# Autodesk Inventor assembly: Lower box main assembly
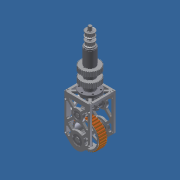
[picture p0: Inventor's stored thumbnail of the model, 180x180]
Saved by Autodesk Inventor 2012 (Build 160160000, 160)
## iProperties
Created: 2012-07-05
Part Number: Lower box main assembly
Document SubType Name: Assembly
Designer: Bryce
Author: Bryce
## Documents named in this file (18)
- C:\Users\Team-2471\Dropbox\Rebound Rumble 2012\Independant Swerves\Inventor 2012\Lower box main assembly.iam
- C:\Users\Team-2471\Dropbox\Rebound Rumble 2012\Independant Swerves\Inventor 2012\lower box side plate.ipt
- C:\Users\Team-2471\Dropbox\Rebound Rumble 2012\Independant Swerves\Inventor 2012\wheel shaft.ipt
- C:\Users\Team-2471\Dropbox\Rebound Rumble 2012\Independant Swerves\Inventor 2012\lower box front plate2.ipt
- C:\Users\Team-2471\Dropbox\Rebound Rumble 2012\Independant Swerves\Imported Components\0.5'' 15 tooth flange.ipt
- C:\Users\Team-2471\Dropbox\Rebound Rumble 2012\Independant Swerves\Inventor 2012\lower box upper shaft.ipt
- C:\Users\Team-2471\Dropbox\Rebound Rumble 2012\Independant Swerves\Inventor 2012\lower box upper plate.ipt
- C:\Users\Team-2471\Dropbox\Rebound Rumble 2012\Independant Swerves\Inventor 2012\vertical drive shaft.ipt
- C:\Users\Team-2471\Dropbox\Rebound Rumble 2012\Independant Swerves\Imported Components\Imported Components\36-5m09-6a4\36-5m09-6a4.ipt
- C:\Users\Team-2471\Dropbox\Rebound Rumble 2012\Independant Swerves\Imported Components\Miter gear.ipt
- C:\Users\Team-2471\Dropbox\Rebound Rumble 2012\Independant Swerves\Inventor 2012\e clip .375in x .039.ipt
- C:\Users\Team-2471\Dropbox\Rebound Rumble 2012\Independant Swerves\Inventor 2012\lower box hub.ipt
- C:\Users\Team-2471\Dropbox\Rebound Rumble 2012\Independant Swerves\Inventor 2012\turn shaft.ipt
- C:\Users\Team-2471\Dropbox\Rebound Rumble 2012\Independant Swerves\Inventor 2012\.375 ID .875 OD bearing.ipt
- C:\Users\Team-2471\Dropbox\Rebound Rumble 2012\Independant Swerves\Imported Components\.375 15 tooth flange short.ipt
- C:\Users\Team-2471\Dropbox\Rebound Rumble 2012\Independant Swerves\Inventor 2012\.5 id 1.125 od flange bearing.ipt
- C:\Users\Team-2471\Dropbox\Rebound Rumble 2012\Independant Swerves\Inventor 2012\new wheel hub.ipt
- C:\Users\Team-2471\Dropbox\Rebound Rumble 2012\Independant Swerves\Inventor 2012\new wheel rim.ipt
## Components (32 placed, 17 different names)
1. wheel shaft:1 — Mate:8, Flush:9, Mate:35, Flush:11, Mate:120, Mate:122, Flush:87, Mate:125, Mate:126, Flush:88, Mate:129
2. lower box front plate2:1 — Mate:113, Mate:114, Flush:78
3. 0.5'' 15 tooth flange:1 — Mate:8, Flush:9, Flush:76, Flush:87
4. lower box upper shaft:1 — Mate:36, Mate:45, Flush:21, Mate:68, Mate:69, Mate:70, Mate:71, Mate:72, Mate:73, Mate:112, Flush:77, Mate:115, Mate:117, Flush:84, Flush:85
5. lower box side plate:2 — Mate:90, Mate:91, Mate:92, Mate:114, Mate:119, Mate:123
6. lower box upper plate:1 — Mate:84, Mate:85, Mate:86, Mate:87, Mate:88, Mate:89, Mate:90, Mate:91, Mate:92, Mate:93, Flush:72, Mate:97, Mate:98, Mate:99, Mate:113, Flush:78
7. lower box front plate2:2 — Mate:87, Mate:88, Mate:89
8. vertical drive shaft:1 — Mate:46, Mate:74, Mate:76, Mate:77, Mate:93, Flush:72, Mate:94, Mate:96, Flush:74, Mate:104, Mate:106, Mate:108, Mate:109, Mate:110, Flush:82, Flush:83, Flush:86
9. lower box side plate:3 — Mate:35, Mate:36, Flush:11, Mate:37, Mate:38, Flush:71, Mate:84, Mate:85, Mate:86, Flush:77, Mate:118, Mate:121
10. 36-5m09-6a4:1 — Mate:96, Flush:75, Flush:81
11. Miter gear:1 — Mate:45, Flush:21, Flush:85
12. Miter gear:2 — Mate:46, Flush:74, Flush:86
13. e clip .375in x .039:1 — Mate:70, Mate:71
14. e clip .375in x .039:2 — Mate:68, Mate:69
15. e clip .375in x .039:3 — Mate:72, Mate:73
16. e clip .375in x .039:4 — Mate:74, Mate:94
17. e clip .375in x .039:5 — Mate:76, Mate:77, Mate:105
18. e clip .375in x .039:6 — Mate:109, Mate:110, Mate:111
19. lower box hub:1 — Mate:97, Mate:98, Mate:99, Mate:100, Flush:73
20. turn shaft:1 — Mate:100, Flush:73, Mate:101, Mate:102, Mate:103, Flush:75, Mate:124, Flush:79, Flush:80, Flush:81
21. .375 ID .875 OD bearing:1 — Mate:101, Mate:102
22. .375 ID .875 OD bearing:2 — Mate:103, Mate:104
23. .375 15 tooth flange short:1 — Mate:108, Mate:111, Flush:82
24. .375 15 tooth flange short:2 — Mate:105, Mate:106, Flush:83
25. .375 15 tooth flange short:3 — Flush:76, Mate:112, Flush:84
26. .375 ID .875 OD bearing:3 — Mate:117, Mate:119
27. .375 ID .875 OD bearing:4 — Mate:115, Mate:118
28. .5 id 1.125 od flange bearing:1 — Mate:120, Mate:121
29. .5 id 1.125 od flange bearing:2 — Mate:122, Mate:123
30. 36-5m09-6a4:2 — Mate:124, Flush:79, Flush:80
31. new wheel hub:1 — Mate:125, Mate:126, Flush:88, Mate:127, Mate:128
32. new wheel rim:1 — Mate:127, Mate:128, Mate:129
## Relationships (80: Mate 59, Flush 21)
- Mate:8: wheel shaft:1 ↔ 0.5'' 15 tooth flange:1
- Flush:9: wheel shaft:1 ↔ 0.5'' 15 tooth flange:1
- Mate:35: wheel shaft:1 ↔ lower box side plate:3
- Mate:36: lower box upper shaft:1 ↔ lower box side plate:3
- Flush:11: wheel shaft:1 ↔ lower box side plate:3
- Mate:37: lower box side plate:3
- Mate:38: lower box side plate:3
- Mate:45: lower box upper shaft:1 ↔ Miter gear:1
- Flush:21: lower box upper shaft:1 ↔ Miter gear:1
- Mate:46: vertical drive shaft:1 ↔ Miter gear:2
- Mate:68: lower box upper shaft:1 ↔ e clip .375in x .039:2
- Mate:69: lower box upper shaft:1 ↔ e clip .375in x .039:2
- Mate:70: lower box upper shaft:1 ↔ e clip .375in x .039:1
- Mate:71: lower box upper shaft:1 ↔ e clip .375in x .039:1
- Mate:72: lower box upper shaft:1 ↔ e clip .375in x .039:3
- Mate:73: lower box upper shaft:1 ↔ e clip .375in x .039:3
- Mate:74: vertical drive shaft:1 ↔ e clip .375in x .039:4
- Mate:76: vertical drive shaft:1 ↔ e clip .375in x .039:5
- Mate:77: vertical drive shaft:1 ↔ e clip .375in x .039:5
- Flush:71: lower box side plate:3
- Mate:84: lower box upper plate:1 ↔ lower box side plate:3
- Mate:85: lower box upper plate:1 ↔ lower box side plate:3
- Mate:86: lower box upper plate:1 ↔ lower box side plate:3
- Mate:87: lower box upper plate:1 ↔ lower box front plate2:2
- Mate:88: lower box upper plate:1 ↔ lower box front plate2:2
- Mate:89: lower box upper plate:1 ↔ lower box front plate2:2
- Mate:90: lower box side plate:2 ↔ lower box upper plate:1
- Mate:91: lower box side plate:2 ↔ lower box upper plate:1
- Mate:92: lower box side plate:2 ↔ lower box upper plate:1
- Mate:93: lower box upper plate:1 ↔ vertical drive shaft:1
- Flush:72 (-25.4 mm): lower box upper plate:1 ↔ vertical drive shaft:1
- Mate:94: vertical drive shaft:1 ↔ e clip .375in x .039:4
- Mate:96: vertical drive shaft:1 ↔ 36-5m09-6a4:1
- Mate:97: lower box upper plate:1 ↔ lower box hub:1
- Mate:98: lower box upper plate:1 ↔ lower box hub:1
- Mate:99: lower box upper plate:1 ↔ lower box hub:1
- Mate:100: lower box hub:1 ↔ turn shaft:1
- Flush:73 (-6.35 mm): lower box hub:1 ↔ turn shaft:1
- Flush:74: vertical drive shaft:1 ↔ Miter gear:2
- Mate:101: turn shaft:1 ↔ .375 ID .875 OD bearing:1
- Mate:102: turn shaft:1 ↔ .375 ID .875 OD bearing:1
- Mate:103: turn shaft:1 ↔ .375 ID .875 OD bearing:2
- Mate:104: vertical drive shaft:1 ↔ .375 ID .875 OD bearing:2
- Mate:105: e clip .375in x .039:5 ↔ .375 15 tooth flange short:2
- Mate:106: vertical drive shaft:1 ↔ .375 15 tooth flange short:2
- Mate:108: vertical drive shaft:1 ↔ .375 15 tooth flange short:1
- Mate:109: vertical drive shaft:1 ↔ e clip .375in x .039:6
- Mate:110: vertical drive shaft:1 ↔ e clip .375in x .039:6
- Mate:111: e clip .375in x .039:6 ↔ .375 15 tooth flange short:1
- Flush:75: 36-5m09-6a4:1 ↔ turn shaft:1
- Flush:76: 0.5'' 15 tooth flange:1 ↔ .375 15 tooth flange short:3
- Mate:112: lower box upper shaft:1 ↔ .375 15 tooth flange short:3
- Flush:77: lower box upper shaft:1 ↔ lower box side plate:3
- Mate:113: lower box front plate2:1 ↔ lower box upper plate:1
- Mate:114: lower box front plate2:1 ↔ lower box side plate:2
- Flush:78: lower box front plate2:1 ↔ lower box upper plate:1
- Mate:115: lower box upper shaft:1 ↔ .375 ID .875 OD bearing:4
- Mate:117: lower box upper shaft:1 ↔ .375 ID .875 OD bearing:3
- Mate:118: lower box side plate:3 ↔ .375 ID .875 OD bearing:4
- Mate:119: lower box side plate:2 ↔ .375 ID .875 OD bearing:3
- Mate:120: wheel shaft:1 ↔ .5 id 1.125 od flange bearing:1
- Mate:121: lower box side plate:3 ↔ .5 id 1.125 od flange bearing:1
- Mate:122: wheel shaft:1 ↔ .5 id 1.125 od flange bearing:2
- Mate:123: lower box side plate:2 ↔ .5 id 1.125 od flange bearing:2
- Mate:124: turn shaft:1 ↔ 36-5m09-6a4:2
- Flush:79: turn shaft:1 ↔ 36-5m09-6a4:2
- Flush:80: turn shaft:1 ↔ 36-5m09-6a4:2
- Flush:81: 36-5m09-6a4:1 ↔ turn shaft:1
- Flush:82: vertical drive shaft:1 ↔ .375 15 tooth flange short:1
- Flush:83: vertical drive shaft:1 ↔ .375 15 tooth flange short:2
- Flush:84: lower box upper shaft:1 ↔ .375 15 tooth flange short:3
- Flush:85: lower box upper shaft:1 ↔ Miter gear:1
- Flush:86: vertical drive shaft:1 ↔ Miter gear:2
- Flush:87: wheel shaft:1 ↔ 0.5'' 15 tooth flange:1
- Mate:125: wheel shaft:1 ↔ new wheel hub:1
- Mate:126: wheel shaft:1 ↔ new wheel hub:1
- Flush:88: wheel shaft:1 ↔ new wheel hub:1
- Mate:127: new wheel hub:1 ↔ new wheel rim:1
- Mate:128: new wheel hub:1 ↔ new wheel rim:1
- Mate:129: wheel shaft:1 ↔ new wheel rim:1
